# Autodesk Inventor assembly: AssemblyV2
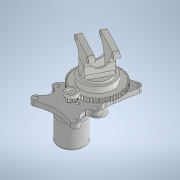
[picture p0: Inventor's stored thumbnail of the model, 180x180]
Saved by Autodesk Inventor 2022 (Build 260153070, 153G)
## iProperties
Created: 2021-10-30
Part Number: AssemblyV2
Document SubType Name: Assembly
Designer: a laptop
Author: a laptop
## Documents named in this file (7)
- C:\Users\a laptop\Desktop\SumoBot\sumobotLIDAR\AssemblyV2.iam
- C:\Users\a laptop\Desktop\SumoBot\sumobotLIDAR\Adapterlowerplate.ipt
- C:\Users\a laptop\Desktop\SumoBot\sumobotLIDAR\MOTOR.ipt
- C:\Users\a laptop\Desktop\SumoBot\sumobotLIDAR\SRM-12-06A.ipt
- C:\Users\a laptop\Desktop\SumoBot\sumobotLIDAR\AssemblyV2\Design Accelerator\Bearing1.iam
- C:\Users\a laptop\Desktop\SumoBot\sumobotLIDAR\sumobotLIDAR\Design Accelerator\Spur Gear12.ipt
- C:\Users\a laptop\Desktop\SumoBot\sumobotLIDAR\sumobotLIDAR\Design Accelerator\Spur Gear23.ipt
## Components (6 placed, 6 different names)
1. Adapterlowerplate:1 — Mate:1, Mate:2, Mate:3, Mate:4, Mate:5, Mate:6, Mate:7, Mate:8, Flush:1
2. MOTOR:1 — Mate:5, Mate:6, Mate:7, Mate:11
3. SRM-12-06A:1 — Mate:1, Mate:2, Mate:3, Mate:4
4. Bearing:1 [sub-assembly] — Mate:8, Flush:1, Mate:9, Mate:10
5. Spur Gear1:1 — Mate:9, Mate:10, Flush:2, Rotation:1
6. Spur Gear2:1 — Flush:2, Mate:11, Rotation:1
## Relationships (14: Mate 11, Flush 2, RelateRotation 1)
- Mate:1: Adapterlowerplate:1 ↔ SRM-12-06A:1
- Mate:2: Adapterlowerplate:1 ↔ SRM-12-06A:1
- Mate:3: Adapterlowerplate:1 ↔ SRM-12-06A:1
- Mate:4: Adapterlowerplate:1 ↔ SRM-12-06A:1
- Mate:5: Adapterlowerplate:1 ↔ MOTOR:1
- Mate:6: Adapterlowerplate:1 ↔ MOTOR:1
- Mate:7: Adapterlowerplate:1 ↔ MOTOR:1
- Mate:8: Adapterlowerplate:1 ↔ Bearing:1
- Flush:1: Adapterlowerplate:1 ↔ Bearing:1
- Mate:9: Bearing:1 ↔ Spur Gear1:1
- Mate:10: Bearing:1 ↔ Spur Gear1:1
- Flush:2: Spur Gear1:1 ↔ Spur Gear2:1
- Mate:11: MOTOR:1 ↔ Spur Gear2:1
- Rotation:1 [RelateRotation] (6 ul): Spur Gear1:1 ↔ Spur Gear2:1
